# Autodesk Inventor assembly: xy-gantry
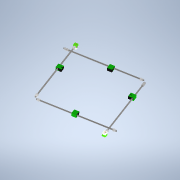
[picture p0: Inventor's stored thumbnail of the model, 180x180]
Saved by Autodesk Inventor 2020.4 (Build 244396000, 396)
## iProperties
Created: 2021-03-01
Part Number: xy-gantry
Document SubType Name: Assembly
Designer: AOB
Mass: 1486.64 g
Surface Area: 1725.8 cm^2
Volume: 269.333 cm^3
Density: 5.51971 g/cm^3
Author: AOB
## Documents named in this file (8)
- C:\Users\marti\Documents\Inventor\ProjectBoron\Boron Ultima\xy-gantry.iam
- C:\Users\marti\Documents\Inventor\ProjectBoron\Boron Ultima\8mm smooth rod.ipt
- C:\Users\marti\Documents\Inventor\ProjectBoron\Boron Ultima\double-head pulley.ipt
- C:\Users\marti\Documents\Inventor\ProjectBoron\Boron Ultima\X-linear bearing shroud.iam
- C:\Users\marti\Documents\Inventor\ProjectBoron\Boron Ultima\Y-linear bearing shroud.iam
- C:\Users\marti\Documents\Inventor\ProjectBoron\Boron Ultima\hotend mount.iam
- C:\Users\marti\Documents\Inventor\ProjectBoron\Boron Ultima\xy-mount-assembly.iam
- C:\Users\marti\Documents\Inventor\ProjectBoron\Boron Ultima\GT2 20T 6mm Powge v2 (1).ipt
## Components (23 placed, 7 different names)
1. xy-mount-assembly:2 [sub-assembly] — Mate:3, Flush:3, Flush:4
2. xy-mount-assembly:3 [sub-assembly] — Mate:1, Mate:2, Flush:5, Flush:6, Mate:21, Mate:19
3. 8mm smooth rod:1 — Mate:2, Mate:4, Flush:5, Mate:16, Mate:25, Mate:9, Flush:8, Flush:10
4. 8mm smooth rod:2 — Mate:1, Mate:3, Flush:4, Flush:6, Mate:19, Mate:27, Mate:12, Flush:7, Flush:13
5. 8mm smooth rod:3 — Mate:6, Mate:8, Flush:1, Flush:3, Mate:10, Mate:22, Mate:24, Flush:12, Mate:52
6. 8mm smooth rod:4 — Mate:5, Mate:7, Flush:2, Mate:11, Mate:17, Mate:26, Flush:11, Flush:9
7. xy-mount-assembly:1 [sub-assembly] — Mate:4, Mate:18
8. xy-mount-assembly:4 [sub-assembly] — Flush:1, Flush:2, Mate:5
9. X-linear bearing shroud:1 [sub-assembly] — Mate:9, Mate:37, Mate:38
10. Y-linear bearing shroud:1 [sub-assembly] — Mate:12, Mate:34
11. Y-linear bearing shroud:2 [sub-assembly] — Mate:11, Mate:35, Mate:36
12. X-linear bearing shroud:2 [sub-assembly] — Mate:10, Mate:39
13. double-head pulley:1 — Mate:16, Mate:21, Flush:8
14. double-head pulley:2 — Mate:17, Mate:18, Flush:9, Mate:26
15. GT2 20T 6mm Powge v2 (1):1 — Flush:7
16. GT2 20T 6mm Powge v2 (1):2 — Mate:22, Mate:6, Mate:52
17. GT2 20T 6mm Powge v2 (1):3 — Mate:27, Flush:13
18. GT2 20T 6mm Powge v2 (1):4 — Mate:7, Flush:11
19. GT2 20T 6mm Powge v2 (1):5 — Mate:24, Mate:8, Flush:12
20. GT2 20T 6mm Powge v2 (1):6 — Mate:25, Flush:10
21. 8mm smooth rod:5 — Mate:34, Mate:35, Mate:36, Mate:46
22. 8mm smooth rod:6 — Mate:37, Mate:38, Mate:39, Mate:47
23. hotend mount:1 [sub-assembly] — Mate:46, Mate:47
## Relationships (50: Mate 37, Flush 13)
- Mate:1: xy-mount-assembly:3 ↔ 8mm smooth rod:2
- Mate:2: xy-mount-assembly:3 ↔ 8mm smooth rod:1
- Mate:3: xy-mount-assembly:2 ↔ 8mm smooth rod:2
- Mate:4: 8mm smooth rod:1 ↔ xy-mount-assembly:1
- Mate:5: 8mm smooth rod:4 ↔ xy-mount-assembly:4
- Mate:6: 8mm smooth rod:3 ↔ GT2 20T 6mm Powge v2 (1):2
- Mate:7: 8mm smooth rod:4 ↔ GT2 20T 6mm Powge v2 (1):4
- Mate:8: 8mm smooth rod:3 ↔ GT2 20T 6mm Powge v2 (1):5
- Flush:1: 8mm smooth rod:3 ↔ xy-mount-assembly:4
- Flush:2: 8mm smooth rod:4 ↔ xy-mount-assembly:4
- Flush:3: xy-mount-assembly:2 ↔ 8mm smooth rod:3
- Flush:4: xy-mount-assembly:2 ↔ 8mm smooth rod:2
- Flush:5: xy-mount-assembly:3 ↔ 8mm smooth rod:1
- Flush:6: xy-mount-assembly:3 ↔ 8mm smooth rod:2
- Mate:10: 8mm smooth rod:3 ↔ X-linear bearing shroud:2
- Mate:11: 8mm smooth rod:4 ↔ Y-linear bearing shroud:2
- Mate:16: 8mm smooth rod:1 ↔ double-head pulley:1
- Mate:17: 8mm smooth rod:4 ↔ double-head pulley:2
- Mate:18 (3 mm): xy-mount-assembly:1 ↔ double-head pulley:2
- Mate:19: xy-mount-assembly:3 ↔ 8mm smooth rod:2
- [Mate] (-3 mm): xy-mount-assembly:3 ↔ GT2 20T 6mm Powge v2 (1):1
- Mate:21 (-3 mm): xy-mount-assembly:3 ↔ double-head pulley:1
- Mate:22: 8mm smooth rod:3 ↔ GT2 20T 6mm Powge v2 (1):2
- [Mate] (3 mm): xy-mount-assembly:2 ↔ GT2 20T 6mm Powge v2 (1):2
- Mate:24: 8mm smooth rod:3 ↔ GT2 20T 6mm Powge v2 (1):5
- Mate:25: 8mm smooth rod:1 ↔ GT2 20T 6mm Powge v2 (1):6
- Mate:26: 8mm smooth rod:4 ↔ double-head pulley:2
- Mate:27: 8mm smooth rod:2 ↔ GT2 20T 6mm Powge v2 (1):3
- [Mate] (3 mm): xy-mount-assembly:4 ↔ GT2 20T 6mm Powge v2 (1):4
- [Mate] (3 mm): xy-mount-assembly:1 ↔ GT2 20T 6mm Powge v2 (1):6
- [Mate] (3 mm): xy-mount-assembly:4 ↔ GT2 20T 6mm Powge v2 (1):5
- [Mate] (3 mm): xy-mount-assembly:2 ↔ GT2 20T 6mm Powge v2 (1):3
- Mate:9: 8mm smooth rod:1 ↔ X-linear bearing shroud:1
- Mate:12: 8mm smooth rod:2 ↔ Y-linear bearing shroud:1
- Mate:34: Y-linear bearing shroud:1 ↔ 8mm smooth rod:5
- Mate:35: Y-linear bearing shroud:2 ↔ 8mm smooth rod:5
- Mate:36: Y-linear bearing shroud:2 ↔ 8mm smooth rod:5
- Mate:37: X-linear bearing shroud:1 ↔ 8mm smooth rod:6
- Mate:38: X-linear bearing shroud:1 ↔ 8mm smooth rod:6
- Mate:39: X-linear bearing shroud:2 ↔ 8mm smooth rod:6
- Mate:46: 8mm smooth rod:5 ↔ hotend mount:1
- Mate:47: 8mm smooth rod:6 ↔ hotend mount:1
- Flush:7 (6 mm): 8mm smooth rod:2 ↔ GT2 20T 6mm Powge v2 (1):1
- Flush:8 (6 mm): 8mm smooth rod:1 ↔ double-head pulley:1
- Flush:9 (-6 mm): 8mm smooth rod:4 ↔ double-head pulley:2
- Flush:10 (6 mm): 8mm smooth rod:1 ↔ GT2 20T 6mm Powge v2 (1):6
- Flush:11 (-6 mm): 8mm smooth rod:4 ↔ GT2 20T 6mm Powge v2 (1):4
- Flush:12 (-6 mm): 8mm smooth rod:3 ↔ GT2 20T 6mm Powge v2 (1):5
- Flush:13 (6 mm): 8mm smooth rod:2 ↔ GT2 20T 6mm Powge v2 (1):3
- Mate:52 (6 mm): 8mm smooth rod:3 ↔ GT2 20T 6mm Powge v2 (1):2
